# Autodesk Inventor assembly: 6138k63
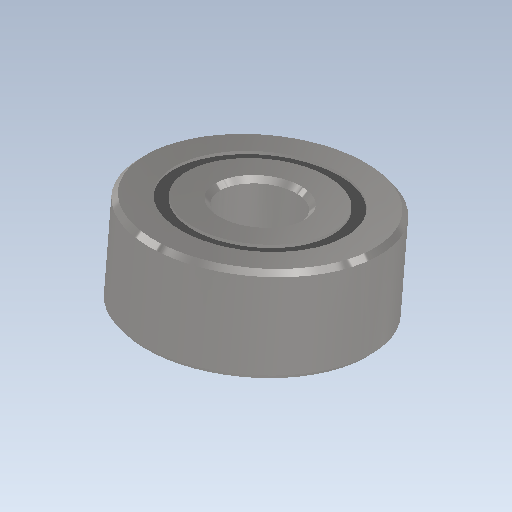
[picture p0: Inventor's stored thumbnail of the model, 512x512]
Saved by Autodesk Inventor 2020.1 (Build 241239000, 239)
## iProperties
Created: 2019-10-27
Part Number: 6138k63
Document SubType Name: Assembly
Designer: agmle
Mass: 1.63848 g
Surface Area: 6.60829 cm^2
Volume: 0.227272 cm^3
Density: 7.20933 g/cm^3
Author: agmle
## Documents named in this file (5)
- M:\documents\Inventor\AutoBuoy\propulsion\bearing\6138k63.iam
- M:\documents\Inventor\AutoBuoy\propulsion\bearing\6138k63_race_inner.ipt
- M:\documents\Inventor\AutoBuoy\propulsion\bearing\6138k63_ball.ipt
- M:\documents\Inventor\AutoBuoy\propulsion\bearing\6138k63_race.ipt
- M:\documents\Inventor\AutoBuoy\propulsion\bearing\6138k63_seal.ipt
## Components (14 placed, 4 different names)
1. 6138k63_race_inner:1 — Cylindrical:1, Tangent:20, Insert:1, Insert:2
2. 6138k63_ball:1 — Tangent:4, Tangent:12, Tangent:13
3. 6138k63_ball:2 — Tangent:3, Tangent:19
4. 6138k63_ball:3 — Tangent:2, Tangent:11, Tangent:12
5. 6138k63_ball:4 — Tangent:1, Tangent:11, Tangent:20
6. 6138k63_ball:5 — Tangent:5, Tangent:18, Tangent:19
7. 6138k63_ball:6 — Tangent:6, Tangent:13, Tangent:14
8. 6138k63_ball:7 — Tangent:7, Tangent:16, Tangent:17
9. 6138k63_ball:8 — Tangent:10, Tangent:17, Tangent:18
10. 6138k63_ball:9 — Tangent:8, Tangent:15, Tangent:16
11. 6138k63_ball:10 — Tangent:9, Tangent:14, Tangent:15
12. 6138k63_race:1 — Tangent:1, Tangent:2, Tangent:3, Tangent:4, Tangent:5, Tangent:6, Tangent:7, Tangent:8, Tangent:9, Tangent:10, Cylindrical:1
13. 6138k63_seal:1 — Insert:2
14. 6138k63_seal:2 — Insert:1
## Relationships (23: Tangent 20, Insert 2, CylindricalJoint 1)
- Tangent:1: 6138k63_ball:4 ↔ 6138k63_race:1
- Tangent:2: 6138k63_ball:3 ↔ 6138k63_race:1
- Tangent:3: 6138k63_ball:2 ↔ 6138k63_race:1
- Tangent:4: 6138k63_ball:1 ↔ 6138k63_race:1
- Tangent:5: 6138k63_ball:5 ↔ 6138k63_race:1
- Tangent:6: 6138k63_ball:6 ↔ 6138k63_race:1
- Tangent:7: 6138k63_ball:7 ↔ 6138k63_race:1
- Tangent:8: 6138k63_ball:9 ↔ 6138k63_race:1
- Tangent:9: 6138k63_ball:10 ↔ 6138k63_race:1
- Tangent:10: 6138k63_ball:8 ↔ 6138k63_race:1
- Tangent:11: 6138k63_ball:3 ↔ 6138k63_ball:4
- Tangent:12: 6138k63_ball:1 ↔ 6138k63_ball:3
- Tangent:13: 6138k63_ball:1 ↔ 6138k63_ball:6
- Tangent:14: 6138k63_ball:6 ↔ 6138k63_ball:10
- Tangent:15: 6138k63_ball:9 ↔ 6138k63_ball:10
- Tangent:16: 6138k63_ball:7 ↔ 6138k63_ball:9
- Tangent:17: 6138k63_ball:7 ↔ 6138k63_ball:8
- Tangent:18: 6138k63_ball:5 ↔ 6138k63_ball:8
- Tangent:19: 6138k63_ball:2 ↔ 6138k63_ball:5
- Cylindrical:1: 6138k63_race_inner:1 ↔ 6138k63_race:1
- Tangent:20: 6138k63_race_inner:1 ↔ 6138k63_ball:4
- Insert:1 (0.0992 mm): 6138k63_race_inner:1 ↔ 6138k63_seal:2
- Insert:2 (0.0992 mm): 6138k63_race_inner:1 ↔ 6138k63_seal:1
